# Autodesk Inventor assembly: Nespresso-Assembly-6x
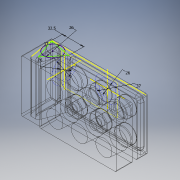
[picture p0: Inventor's stored thumbnail of the model, 180x180]
Saved by Autodesk Inventor 2017 (Build 210142000, 142)
## iProperties
Created: 2018-11-11
Part Number: Nespresso-Assembly-6x
Document SubType Name: Assembly
Designer: 45027374
Author: 45027374
## Documents named in this file (5)
- C:\cloudstor\Documents\3Dprints\nespresso-speedfiller\Nespresso-Assembly-6x.iam
- C:\cloudstor\Documents\3Dprints\nespresso-speedfiller\NespressoSpeedfiller-6x-long-base.ipt
- C:\cloudstor\Documents\3Dprints\nespresso-speedfiller\NespressoSpeedfiller-6X-long.ipt
- C:\cloudstor\Documents\3Dprints\nespresso-speedfiller\NespressoSpeedfiller-6X-long-tamper.ipt
- C:\cloudstor\Documents\3Dprints\nespresso-speedfiller\NespressoSpeedfiller-6X-long-scraper.ipt
## Components (4 placed, 4 different names)
1. NespressoSpeedfiller-6x-long-base:1 — Mate:1, Mate:2, Mate:3, Mate:4, Mate:5
2. NespressoSpeedfiller-6X-long:1 — Mate:4, Mate:5, Mate:6, Mate:7
3. NespressoSpeedfiller-6X-long-tamper:1 — Mate:6, Mate:7
4. NespressoSpeedfiller-6X-long-scraper:1
## Relationships (7: Mate 7)
- Mate:1: NespressoSpeedfiller-6x-long-base:1
- Mate:2: NespressoSpeedfiller-6x-long-base:1
- Mate:3: NespressoSpeedfiller-6x-long-base:1
- Mate:4: NespressoSpeedfiller-6x-long-base:1 ↔ NespressoSpeedfiller-6X-long:1
- Mate:5: NespressoSpeedfiller-6x-long-base:1 ↔ NespressoSpeedfiller-6X-long:1
- Mate:6: NespressoSpeedfiller-6X-long:1 ↔ NespressoSpeedfiller-6X-long-tamper:1
- Mate:7: NespressoSpeedfiller-6X-long:1 ↔ NespressoSpeedfiller-6X-long-tamper:1
